# Autodesk Inventor assembly: wheel_set
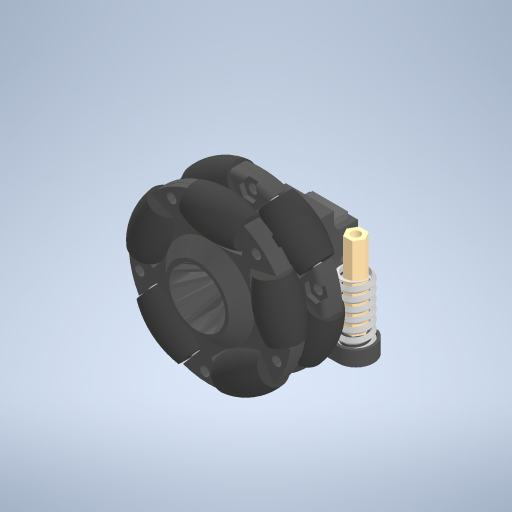
[picture p0: Inventor's stored thumbnail of the model, 512x512]
Saved by Autodesk Inventor 2024.1 (Build 281209000, 209)
## iProperties
Created: 2024-12-19
Part Number: wheel_set
Document SubType Name: Assembly
Designer: hibik
Author: hibik
## Documents named in this file (6)
- C:\Users\hibik\Documents\Robomech\RESCUE\ORCA\hard\omni_wheel\Assy_omni_wheel.iam
- C:\Users\hibik\Documents\Robomech\RESCUE\ORCA\hard\omni_wheel\Assy_motor.iam
- C:\Users\hibik\Documents\Robomech\RESCUE\ORCA\hard\omni_wheel\Assy_wheel.iam
- C:\Users\hibik\Documents\Robomech\RESCUE\ORCA\hard\std_parts\bearing_3_6_2.5.ipt
- C:\Users\hibik\Documents\Robomech\RESCUE\ORCA\hard\std_parts\spring_pi10_23.ipt
- C:\Users\hibik\Documents\Robomech\RESCUE\ORCA\hard\omni_wheel\spacer.ipt
## Components (10 placed, 5 different names)
1. Assy_motor:1 [sub-assembly] — 挿入:1, 挿入:2, 挿入:3, 挿入:4, 挿入:5, 挿入:6, 挿入:7, 挿入:8, 挿入:9, 角度:1, 角度:2
2. Assy_wheel:1 [sub-assembly] — 挿入:5
3. bearing_3_6_2.5:1 — 挿入:1
4. bearing_3_6_2.5:2 — 挿入:2
5. bearing_3_6_2.5:3 — 挿入:3
6. bearing_3_6_2.5:4 — 挿入:4
7. spring_pi10_23:1 — 挿入:7
8. spring_pi10_23:2 — 挿入:6
9. spacer:1 — 挿入:9, 角度:1
10. spacer:2 — 挿入:8, 角度:2
## Relationships (11: Insert 9, Angle 2)
- 挿入:1 [Insert]: Assy_motor:1 ↔ bearing_3_6_2.5:1
- 挿入:2 [Insert]: Assy_motor:1 ↔ bearing_3_6_2.5:2
- 挿入:3 [Insert]: Assy_motor:1 ↔ bearing_3_6_2.5:3
- 挿入:4 [Insert]: Assy_motor:1 ↔ bearing_3_6_2.5:4
- 挿入:5 [Insert]: Assy_motor:1 ↔ Assy_wheel:1
- 挿入:6 [Insert]: Assy_motor:1 ↔ spring_pi10_23:2
- 挿入:7 [Insert]: Assy_motor:1 ↔ spring_pi10_23:1
- 挿入:8 [Insert]: Assy_motor:1 ↔ spacer:2
- 挿入:9 [Insert]: Assy_motor:1 ↔ spacer:1
- 角度:1 [Angle] (0 deg): Assy_motor:1 ↔ spacer:1
- 角度:2 [Angle] (0 deg): Assy_motor:1 ↔ spacer:2
